# Autodesk Inventor assembly: s-assy-unit-j3.0093
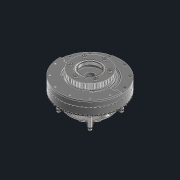
[picture p0: Inventor's stored thumbnail of the model, 180x180]
Saved by Autodesk Inventor 2022 (Build 260153000, 153)
## iProperties
Created: 2021-07-12
Document SubType Name: Assembly
Designer: yuta0
Mass: 948.024 g
Surface Area: 2842.47 cm^2
Volume: 426.271 cm^3
Density: 2.224 g/cm^3
Author: yuta0
## Documents named in this file (8)
- C:\Users\yuta0\Documents\GitHub\catchrobo_hardware\assy-robot\s-assy-unit-j3.iam
- C:\Users\yuta0\Documents\GitHub\catchrobo_hardware\assy-robot\s-assy-sun_gear.iam
- C:\Users\yuta0\Documents\GitHub\catchrobo_hardware\assy-robot\s-assy-unit-j2-2-gear.iam
- C:\Users\yuta0\Documents\GitHub\catchrobo_hardware\assy-robot\base13.ipt
- C:\Users\yuta0\Documents\GitHub\catchrobo_hardware\assy-robot\s-assy-ring_gear.iam
- C:\Users\yuta0\Documents\GitHub\catchrobo_hardware\assy-robot\steel_plate2.ipt
- C:\Users\yuta0\Documents\GitHub\catchrobo_hardware\assy-robot\B6808ZZ.ipt
- C:\Users\yuta0\Documents\GitHub\catchrobo_hardware\assy-robot\CB4-30.ipt
## Components (12 placed, 7 different names)
1. s-assy-sun_gear:1 [sub-assembly] — メイト:1, メイト:2, メイト:66
2. s-assy-unit-j2-2-gear:1 [sub-assembly] — メイト:1, フラッシュ:1, メイト:2, メイト:49, メイト:51, メイト:52, メイト:53, メイト:64
3. base13:1 — メイト:49, メイト:51, メイト:61, メイト:62, メイト:63, メイト:64
4. s-assy-ring_gear:1 [sub-assembly] — メイト:52, メイト:53, メイト:59, メイト:60, メイト:65, メイト:66
5. steel_plate2:1 — メイト:59, メイト:60, メイト:65
6. B6808ZZ:1 — メイト:61, メイト:62
7. CB4-30:1 — メイト:63
8. CB4-30:2
9. CB4-30:3
10. CB4-30:4
11. CB4-30:5
12. CB4-30:6
## Component patterns: (6 elements, first: CB4-30:1)
## Relationships (16: Mate 15, Flush 1)
- メイト:1 [Mate]: s-assy-sun_gear:1 ↔ s-assy-unit-j2-2-gear:1
- フラッシュ:1 [Flush]: s-assy-unit-j2-2-gear:1
- メイト:2 [Mate]: s-assy-sun_gear:1 ↔ s-assy-unit-j2-2-gear:1
- メイト:49 [Mate]: s-assy-unit-j2-2-gear:1 ↔ base13:1
- メイト:51 [Mate]: s-assy-unit-j2-2-gear:1 ↔ base13:1
- メイト:52 [Mate]: s-assy-unit-j2-2-gear:1 ↔ s-assy-ring_gear:1
- メイト:53 [Mate]: s-assy-unit-j2-2-gear:1 ↔ s-assy-ring_gear:1
- [Mate]: base13:1 ↔ CB4-30:1
- メイト:59 [Mate]: s-assy-ring_gear:1 ↔ steel_plate2:1
- メイト:60 [Mate]: s-assy-ring_gear:1 ↔ steel_plate2:1
- メイト:61 [Mate]: base13:1 ↔ B6808ZZ:1
- メイト:62 [Mate]: base13:1 ↔ B6808ZZ:1
- メイト:63 [Mate]: base13:1 ↔ CB4-30:1
- メイト:64 [Mate]: s-assy-unit-j2-2-gear:1 ↔ base13:1
- メイト:65 [Mate]: s-assy-ring_gear:1 ↔ steel_plate2:1
- メイト:66 [Mate]: s-assy-sun_gear:1 ↔ s-assy-ring_gear:1
